# Autodesk Inventor assembly: Beebox_ass
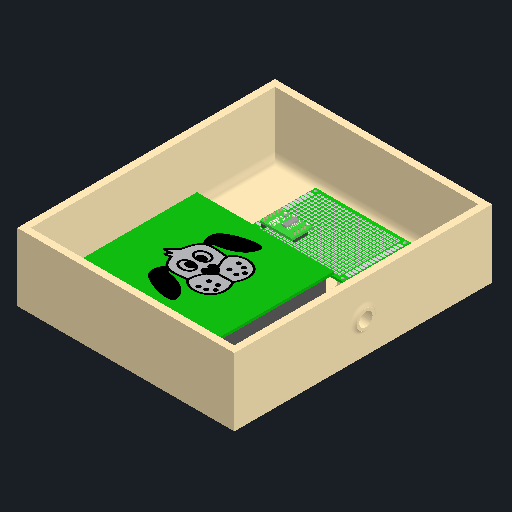
[picture p0: Inventor's stored thumbnail of the model, 512x512]
Saved by Autodesk Inventor 2027 (Build 310192060, 192F)
## iProperties
Created: 2026-10-02
Part Number: Beebox_ass
Document SubType Name: Assembly
Designer: notra
Author: notra
## Documents named in this file (5)
- C:\Users\notra\Desktop\BeeBox\3dFiles\Beebox_ass.iam
- C:\Users\notra\Desktop\BeeBox\3dFiles\CaseBitDog.ipt
- C:\Users\notra\Desktop\BeeBox\3dFiles\Bitdoglab.ipt
- C:\Users\notra\Desktop\BeeBox\3dFiles\pcb_5x7\pcb_5x7.ipt
- C:\Users\notra\Downloads\Assembly7.iam
## Components (4 placed, 4 different names)
1. CaseBitDog:1 — Mate:1, Flush:1, Flush:2, Mate:2, Flush:3, Flush:4
2. Bitdoglab:1 — Mate:2, Flush:3, Flush:4
3. pcb_5x7:1 — Mate:1, Flush:1, Flush:2, Mate:3, Flush:5, Flush:6
4. Assembly7:1 [sub-assembly] — Mate:3, Flush:5, Flush:6
## Relationships (9: Flush 6, Mate 3)
- Mate:1: CaseBitDog:1 ↔ pcb_5x7:1
- Flush:1: CaseBitDog:1 ↔ pcb_5x7:1
- Flush:2: CaseBitDog:1 ↔ pcb_5x7:1
- Mate:2: CaseBitDog:1 ↔ Bitdoglab:1
- Flush:3: CaseBitDog:1 ↔ Bitdoglab:1
- Flush:4 (-10 mm): CaseBitDog:1 ↔ Bitdoglab:1
- Mate:3: pcb_5x7:1 ↔ Assembly7:1
- Flush:5 (4.55 mm): pcb_5x7:1 ↔ Assembly7:1
- Flush:6 (4.2 mm): pcb_5x7:1 ↔ Assembly7:1
